# Autodesk Inventor assembly: motor_1608
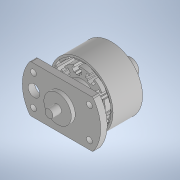
[picture p0: Inventor's stored thumbnail of the model, 180x180]
Saved by Autodesk Inventor 2020 (Build 240168000, 168)
## iProperties
Created: 2020-01-30
Part Number: motor_1608
Document SubType Name: Assembly
Designer: psrobotics
Author: psrobotics
## Documents named in this file (3)
- D:\projects-3\haptic hand gen2\hardware\tip_engine_1\motor_1608.iam
- D:\projects-3\haptic hand gen2\hardware\tip_engine_1\motor_1608_inner.ipt
- D:\projects-3\haptic hand gen2\hardware\tip_engine_1\motor_1608_outer.ipt
## Components (2 placed, 2 different names)
1. motor_1608_inner:1 — Insert:1, Angle:1
2. motor_1608_outer:1 — Insert:1, Angle:1
## Relationships (2: Insert 1, Angle 1)
- Insert:1 (3.5 mm): motor_1608_inner:1 ↔ motor_1608_outer:1
- Angle:1 (0 deg): motor_1608_inner:1 ↔ motor_1608_outer:1
